# Autodesk Inventor assembly: Rotor
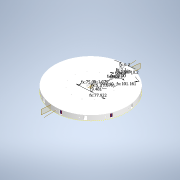
[picture p0: Inventor's stored thumbnail of the model, 180x180]
Saved by Autodesk Inventor 2022.2 (Build 262287000, 287)
## iProperties
Created: 2022-07-21
Part Number: Rotor
Document SubType Name: Assembly
Designer: ABL
Author: ABL
## Documents named in this file (7)
- C:\GitHubRepos\PHYS-12-Website\content\portfolio\Final Project\CAD\Rotor.iam
- C:\GitHubRepos\PHYS-12-Website\content\portfolio\Final Project\CAD\RotorBody.ipt
- C:\GitHubRepos\PHYS-12-Website\content\portfolio\Final Project\CAD\DriveMagnet.ipt
- C:\GitHubRepos\PHYS-12-Website\content\portfolio\Final Project\CAD\HalbachMagnet.ipt
- C:\GitHubRepos\PHYS-12-Website\content\portfolio\Final Project\CAD\SensorMagnet.ipt
- C:\GitHubRepos\PHYS-12-Website\content\portfolio\Final Project\CAD\HalbachMagnet_MIR.ipt
- C:\GitHubRepos\PHYS-12-Website\content\portfolio\Final Project\CAD\MotorGlobalParameters.xlsx
## Components (43 placed, 5 different names)
1. RotorBody:1 — Mate:1, Mate:2, Mate:3, Mate:4, Flush:7, Mate:5, Mate:7, Mate:8, Mate:9, Angle:1
2. SensorMagnet:1 — Mate:7, Mate:8
3. SensorMagnet:2
4. SensorMagnet:3
5. SensorMagnet:4
6. SensorMagnet:5
7. SensorMagnet:6
8. DriveMagnet:1 — Mate:1, Mate:2, Mate:3
9. DriveMagnet:2
10. HalbachMagnet:1 — Mate:4, Flush:7, Mate:5
11. HalbachMagnet:2
12. DriveMagnet:3
13. DriveMagnet:4
14. HalbachMagnet:3
15. HalbachMagnet:4
16. DriveMagnet:5
17. DriveMagnet:6
18. HalbachMagnet:5
19. HalbachMagnet:6
20. DriveMagnet:7
21. DriveMagnet:8
22. HalbachMagnet:7
23. HalbachMagnet:8
24. DriveMagnet:9
25. DriveMagnet:10
26. HalbachMagnet:9
27. HalbachMagnet:10
28. DriveMagnet:11
29. DriveMagnet:12
30. HalbachMagnet:11
31. HalbachMagnet:12
32. HalbachMagnet_MIR:1
33. HalbachMagnet_MIR:2
34. HalbachMagnet_MIR:3
35. HalbachMagnet_MIR:4
36. HalbachMagnet_MIR:5
37. HalbachMagnet_MIR:6
38. HalbachMagnet_MIR:7
39. HalbachMagnet_MIR:8
40. HalbachMagnet_MIR:9
41. HalbachMagnet_MIR:10
42. HalbachMagnet_MIR:11
43. HalbachMagnet_MIR:12
## Component patterns: NorthMagnets (6 elements), SouthMagnets (6 elements), DriveMagnetStack (2 elements), HalbachMagnetStack (2 elements), DriveMagnetStack:2 (2 elements), HalbachMagnetStack:2 (2 elements), DriveMagnetStack:3 (2 elements), HalbachMagnetStack:3 (2 elements), DriveMagnetStack:4 (2 elements), HalbachMagnetStack:4 (2 elements), DriveMagnetStack:5 (2 elements), HalbachMagnetStack:5 (2 elements), DriveMagnetStack:6 (2 elements), HalbachMagnetStack:6 (2 elements), SouthHalbachMagnet (2 elements), SouthHalbachMagnet:2 (2 elements), SouthHalbachMagnet:3 (2 elements), SouthHalbachMagnet:4 (2 elements), SouthHalbachMagnet:5 (2 elements), SouthHalbachMagnet:6 (2 elements)
## Relationships (10: Mate 8, Flush 1, Angle 1)
- Mate:1: RotorBody:1 ↔ DriveMagnet:1
- Mate:2 (0.1 mm): RotorBody:1 ↔ DriveMagnet:1
- Mate:3 (0.1 mm): RotorBody:1 ↔ DriveMagnet:1
- Mate:4 (0.1 mm): RotorBody:1 ↔ HalbachMagnet:1
- Flush:7 (0.1 mm): RotorBody:1 ↔ HalbachMagnet:1
- Mate:5: RotorBody:1 ↔ HalbachMagnet:1
- Mate:7: RotorBody:1 ↔ SensorMagnet:1
- Mate:8: RotorBody:1 ↔ SensorMagnet:1
- Mate:9: RotorBody:1
- Angle:1 (90 deg): RotorBody:1
## Named parameters: gap = 0.1 mm, airgap = 0.4 mm, driveMagnet_length = 60 mm, driveMagnet_width = 10 mm, driveMagnet_height = 5 mm, halbachMagnet_length = 60 mm, halbachMagnet_width = 10 mm, halbachMagnet_height = 3 mm, sensorMagnet_diameter = 5 mm, sensorMagnet_height = 2.66667 mm, numMagnetSets = 12, numElectromagnets = 9, wallgap = 2 mm, halbachMagnet_numStacked = 2, driveMagnet_centerSpacingRadius = 38.96113 mm, motorRadius = 103.16113 mm, rotorThickness = 14.1 mm, driveMagnet_numStacked = 2, shaftDiameter = 8 mm, flangeBearing_outerDiameter = 16 mm, flangeBearing_innerDiameter = 8 mm, flangeBearing_height = 5 mm, flangeBearing_flangeHeight = 1 mm, flangeBearing_flangeDiameter = 18 mm, magnetTrapNut_height = 1.2 mm, magnetTrapNut_sideToSide = 4 mm, magnetTrapBolt_headHeight = 2 mm, magnetTrapBolt_headDiameter = 3.98 mm, magnetTrapBolt_diameter = 2 mm, statorThickness = 16 mm, rotor_mountingLipHeight = 8 mm, magnetTrapBolt_shaftLength = 20 mm, magnetTrapHexNut_sideToSide = 4 mm, magnetTrapSquareNut_sideLength = 4 mm, magnetTrapSquareNut_height = 1.2 mm, magnetTrapHexNut_height = 1.2 mm, magnetTrap_wingDegrees = 4.443207 deg, magnetTrap_wingOuterDegrees = 11.764706 deg, rotorRadius = 101.16113 mm, rotorBandSquareNut_sideLength = 4 mm, rotorBandHexNut_height = 1.2 mm, rotorBandBolt_shaftLength = 20 mm, rotorBandHexNut_sideToSide = 4 mm, rotorBandSquareNut_height = 1.2 mm, rotorBandBolt_headHeight = 2 mm, rotorBandBolt_headDiameter = 3.98 mm, rotorBandBolt_diameter = 2 mm, rotorBandThickness = 4.1 mm, shaftLength = 200 mm, flangeCoupling_collarOuterDiameter = 16 mm, flangeCoupling_flangeHoleEdgeToEdge = 2.05 mm, flangeCoupling_innerDiameter = 8 mm, flangeCoupling_flangeHoleDiameter = 3.9 mm, flangeCoupling_flangeHeight = 3.1 mm, flangeCoupling_collarHeight = 10 mm, flangeCoupling_flangeDiameter = 32 mm, flangeCoupling_height = 13.1 mm, flangeCoupling_mountHoleDiameter = 3.9 mm, flangeCoupling_mountHoleEdgeToEdge = 2.05 mm, statorRadius = 99.16113 mm, coilThickness = 12 mm, statorMountBolt_diameter = 4 mm, statorMountBolt_headDiameter = 7 mm, statorMountBolt_headHeight = 4 mm, statorMountBolt_shaftLength = 17.1 mm, statorMountHexNut_height = 4 mm, statorMountHexNut_sideToSide = 8 mm, sensorMagnet_ringRadius = 23.48057 mm, coil_percentCoverage = 0.6, statorSpokeDegrees = 4 deg, coil_bulge = 3 mm, coil_cornerRadius = 10 mm, coil_width = 10 mm, statorCoilBolt_shaftLength = 12 mm, statorCoilHexNut_height = 1.2 mm, statorCoilBolt_headHeight = 2 mm, statorCoilBolt_diameter = 2 mm, statorCoilBolt_headDiameter = 3.98 mm, statorCoilHexNut_sideToSide = 4 mm
